# Autodesk Inventor assembly: Behavioural Device assembly 2
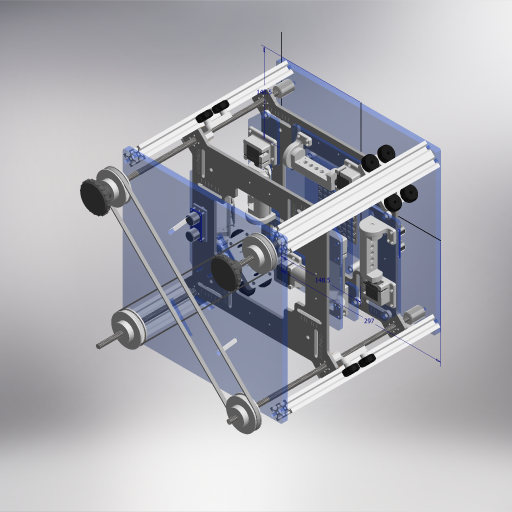
[picture p0: Inventor's stored thumbnail of the model, 512x512]
Saved by Autodesk Inventor 2023 (Build 270158000, 158)
## iProperties
Created: 2020-08-17
Part Number: Behavioural Device assembly 2
Document SubType Name: Assembly
Designer: ferrerx
Author: ferrerx
## iProperties of the stored document MemberDocs/xAaaaqbcaAaaaaaaaAaaaqxjcCb
Created: 2020-08-17
Part Number: Behavioural Device assembly 2
Document SubType Name: Assembly
Designer: ferrerx
Author: ferrerx
## Documents named in this file (26)
- C:\Users\ferrerx\Documents\GitHub\OptoPi\OptoPi V1\Mechanical components\Design files\Inventor Assembly\Behavioural Device assembly 2.iam
- C:\Users\ferrerx\Desktop\Projects\Prieto-Godino Lab\Drosophila Larvae Behavioural Device\Device design V4\Inventor Assembly\aluminum profile.ipt
- C:\Users\ferrerx\Desktop\Projects\Prieto-Godino Lab\Drosophila Larvae Behavioural Device\Device design V4\Inventor Assembly\Z stage Base.ipt
- C:\Users\ferrerx\Desktop\Projects\Prieto-Godino Lab\Drosophila Larvae Behavioural Device\Device design V4\Inventor Assembly\Big pulley.ipt
- C:\Users\ferrerx\Desktop\Projects\Prieto-Godino Lab\Drosophila Larvae Behavioural Device\Device design V4\Inventor Assembly\Shaft connector.ipt
- C:\Users\ferrerx\Desktop\Projects\Prieto-Godino Lab\Drosophila Larvae Behavioural Device\Device design V4\Inventor Assembly\Lead screw.ipt
- C:\Users\ferrerx\Desktop\Projects\Prieto-Godino Lab\Drosophila Larvae Behavioural Device\Device design V4\Inventor Assembly\Lead screw manual adjuster.ipt
- C:\Users\ferrerx\Desktop\Projects\Prieto-Godino Lab\Drosophila Larvae Behavioural Device\Device design V4\Inventor Assembly\Z stage Roof 2.ipt
- C:\Users\ferrerx\Desktop\Projects\Prieto-Godino Lab\Drosophila Larvae Behavioural Device\Device design V4\Inventor Assembly\Belt.ipt
- C:\Users\ferrerx\Desktop\Projects\Prieto-Godino Lab\Drosophila Larvae Behavioural Device\Device design V4\Inventor Assembly\Arena assembly.iam
- C:\Users\ferrerx\Desktop\Projects\Prieto-Godino Lab\Drosophila Larvae Behavioural Device\Device design V4\Inventor Assembly\Platform assembly with IR.iam
- C:\Users\ferrerx\Desktop\Projects\Prieto-Godino Lab\Drosophila Larvae Behavioural Device\Device design V4\Inventor Assembly\Platform RGB assembly.iam
- C:\Users\ferrerx\Desktop\Projects\Prieto-Godino Lab\Drosophila Larvae Behavioural Device\Device design V4\Inventor Assembly\Camera stage V2\Camera stage V2 assembly.iam
- C:\Users\ferrerx\Documents\GitHub\OptoPi\OptoPi V1\Mechanical components\Design files\Inventor Assembly\aluminum profile.ipt
- C:\Users\ferrerx\Documents\GitHub\OptoPi\OptoPi V1\Mechanical components\Design files\Inventor Assembly\Z stage Base.ipt
- C:\Users\ferrerx\Documents\GitHub\OptoPi\OptoPi V1\Mechanical components\Design files\Inventor Assembly\Big pulley.ipt
- C:\Users\ferrerx\Documents\GitHub\OptoPi\OptoPi V1\Mechanical components\Design files\Inventor Assembly\Shaft connector.ipt
- C:\Users\ferrerx\Documents\GitHub\OptoPi\OptoPi V1\Mechanical components\Design files\Inventor Assembly\Lead screw.ipt
- C:\Users\ferrerx\Documents\GitHub\OptoPi\OptoPi V1\Mechanical components\Design files\Inventor Assembly\Lead screw manual adjuster.ipt
- C:\Users\ferrerx\Documents\GitHub\OptoPi\OptoPi V1\Mechanical components\Design files\Inventor Assembly\Z stage Roof 2.ipt
- C:\Users\ferrerx\Documents\GitHub\OptoPi\OptoPi V1\Mechanical components\Design files\Inventor Assembly\Belt.ipt
- C:\Users\ferrerx\Documents\GitHub\OptoPi\OptoPi V1\Mechanical components\Design files\Inventor Assembly\Arena assembly.iam
- C:\Users\ferrerx\Documents\GitHub\OptoPi\OptoPi V1\Mechanical components\Design files\Inventor Assembly\Platform assembly with IR.iam
- C:\Users\ferrerx\Documents\GitHub\OptoPi\OptoPi V1\Mechanical components\Design files\Inventor Assembly\Platform RGB assembly.iam
- C:\Users\ferrerx\Documents\GitHub\OptoPi\OptoPi V1\Mechanical components\Design files\Inventor Assembly\Camera stage V2\Camera stage V2 assembly.iam
- C:\Users\ferrerx\Desktop\Projects\Prieto-Godino Lab\Drosophila Larvae Behavioural Device\Device design V4\Inventor Assembly\Behavioural Device assembly 2.iam
## Components (26 placed, 12 different names)
1. aluminum profile:1 — Mate:7, Mate:8, Mate:9, Mate:102, Mate:103, Mate:104, Mate:338, Mate:339, Mate:340
2. aluminum profile:2 — Mate:1, Mate:2, Mate:3, Angle:1
3. Z stage Base:2 — Mate:1, Mate:2, Mate:3, Mate:4, Mate:5, Mate:6, Mate:7, Mate:8, Mate:9, Mate:10, Mate:11, Mate:12, Mate:75, Mate:76, Mate:77, Mate:78, Mate:145, Mate:146, Mate:147, Mate:148, Mate:328
4. aluminum profile:3 — Mate:10, Mate:11, Mate:12
5. aluminum profile:4 — Mate:4, Mate:5, Mate:6, Angle:2
6. Big pulley:1 — Mate:95, Mate:106
7. Big pulley:2 — Mate:94, Mate:105, Mate:251, Mate:252
8. Shaft connector:1 — Mate:75, Mate:76, Mate:79, Mate:81
9. Shaft connector:2 — Mate:77, Mate:78, Mate:82, Mate:83
10. Lead screw:3 — Mate:79, Mate:81, Mate:94, Mate:99, Mate:100, Mate:336
11. Lead screw:4 — Mate:82, Mate:83, Mate:95
12. Lead screw manual adjuster:2 — Mate:99, Mate:100
13. Z stage Roof 2:1 — Mate:102, Mate:103, Mate:104, Mate:105, Mate:106
14. Lead screw:5 — Mate:149, Mate:151, Mate:154, Mate:156, Mate:157
15. Lead screw:6 — Mate:150, Mate:152, Mate:153, Mate:337
16. Lead screw manual adjuster:3 — Mate:156, Mate:157, Mate:160
17. Big pulley:3 — Mate:154, Mate:160, Mate:253, Mate:254
18. Big pulley:4 — Mate:153
19. Shaft connector:3 — Mate:145, Mate:148, Mate:150, Mate:152
20. Shaft connector:4 — Mate:146, Mate:147, Mate:149, Mate:151
21. Belt:1 — Mate:251, Mate:252
22. Belt:2 — Mate:253, Mate:254
23. Arena assembly:1 [sub-assembly] — Mate:328
24. Platform assembly with IR:1 [sub-assembly] — Mate:336, Angle:1
25. Platform RGB assembly:1 [sub-assembly] — Mate:337, Angle:2
26. Camera stage V2 assembly:1 [sub-assembly] — Mate:338, Mate:339, Mate:340
## Relationships (54: Mate 52, Angle 2)
- Mate:1: aluminum profile:2 ↔ Z stage Base:2
- Mate:2: aluminum profile:2 ↔ Z stage Base:2
- Mate:3: aluminum profile:2 ↔ Z stage Base:2
- Mate:4: Z stage Base:2 ↔ aluminum profile:4
- Mate:5: Z stage Base:2 ↔ aluminum profile:4
- Mate:6: Z stage Base:2 ↔ aluminum profile:4
- Mate:7: aluminum profile:1 ↔ Z stage Base:2
- Mate:8: aluminum profile:1 ↔ Z stage Base:2
- Mate:9: aluminum profile:1 ↔ Z stage Base:2
- Mate:10: Z stage Base:2 ↔ aluminum profile:3
- Mate:11: Z stage Base:2 ↔ aluminum profile:3
- Mate:12: Z stage Base:2 ↔ aluminum profile:3
- Mate:75: Z stage Base:2 ↔ Shaft connector:1
- Mate:76: Z stage Base:2 ↔ Shaft connector:1
- Mate:77: Z stage Base:2 ↔ Shaft connector:2
- Mate:78: Z stage Base:2 ↔ Shaft connector:2
- Mate:79: Shaft connector:1 ↔ Lead screw:3
- Mate:81: Shaft connector:1 ↔ Lead screw:3
- Mate:82: Shaft connector:2 ↔ Lead screw:4
- Mate:83: Shaft connector:2 ↔ Lead screw:4
- Mate:94: Big pulley:2 ↔ Lead screw:3
- Mate:95: Big pulley:1 ↔ Lead screw:4
- Mate:99: Lead screw:3 ↔ Lead screw manual adjuster:2
- Mate:100: Lead screw:3 ↔ Lead screw manual adjuster:2
- Mate:102: aluminum profile:1 ↔ Z stage Roof 2:1
- Mate:103: aluminum profile:1 ↔ Z stage Roof 2:1
- Mate:104: aluminum profile:1 ↔ Z stage Roof 2:1
- Mate:105: Big pulley:2 ↔ Z stage Roof 2:1
- Mate:106: Big pulley:1 ↔ Z stage Roof 2:1
- Mate:145: Z stage Base:2 ↔ Shaft connector:3
- Mate:146: Z stage Base:2 ↔ Shaft connector:4
- Mate:147: Z stage Base:2 ↔ Shaft connector:4
- Mate:148: Z stage Base:2 ↔ Shaft connector:3
- Mate:149: Lead screw:5 ↔ Shaft connector:4
- Mate:150: Lead screw:6 ↔ Shaft connector:3
- Mate:151: Lead screw:5 ↔ Shaft connector:4
- Mate:152: Lead screw:6 ↔ Shaft connector:3
- Mate:153: Lead screw:6 ↔ Big pulley:4
- Mate:154: Lead screw:5 ↔ Big pulley:3
- Mate:156: Lead screw:5 ↔ Lead screw manual adjuster:3
- Mate:157: Lead screw:5 ↔ Lead screw manual adjuster:3
- Mate:160: Lead screw manual adjuster:3 ↔ Big pulley:3
- Mate:251: Big pulley:2 ↔ Belt:1
- Mate:252 (1 mm): Big pulley:2 ↔ Belt:1
- Mate:253: Big pulley:3 ↔ Belt:2
- Mate:254 (1 mm): Big pulley:3 ↔ Belt:2
- Mate:328: Z stage Base:2 ↔ Arena assembly:1
- Mate:336: Lead screw:3 ↔ Platform assembly with IR:1
- Angle:1 (0 deg): aluminum profile:2 ↔ Platform assembly with IR:1
- Mate:337: Lead screw:6 ↔ Platform RGB assembly:1
- Angle:2 (0 deg): aluminum profile:4 ↔ Platform RGB assembly:1
- Mate:338: aluminum profile:1 ↔ Camera stage V2 assembly:1
- Mate:339: aluminum profile:1 ↔ Camera stage V2 assembly:1
- Mate:340: aluminum profile:1 ↔ Camera stage V2 assembly:1
